# Autodesk Inventor assembly: final-print-(with_numbar)
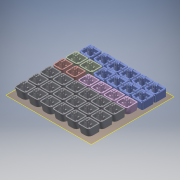
[picture p0: Inventor's stored thumbnail of the model, 180x180]
Saved by Autodesk Inventor 2018 (Build 220112000, 112)
## iProperties
Created: 2017-07-27
Part Number: final-print-(with_numbar)
Document SubType Name: Assembly
Designer: Jason Cemra
Author: Jason Cemra
## Documents named in this file (4)
- C:\Users\Jason Cemra\Documents\Logical Store\StenoToppers\stenotoppers\cherrymx\print-assemblies\final-print-(with_numbar).iam
- C:\Users\Jason Cemra\Documents\Logical Store\StenoToppers\stenotoppers\cherrymx\print-assemblies\final-print.iam
- C:\Users\Jason Cemra\Documents\Logical Store\StenoToppers\stenotoppers\cherrymx\stenotoppers\numbar_cmx.ipt
- C:\Users\Jason Cemra\Documents\Logical Store\StenoToppers\stenotoppers\cherrymx\stenotoppers.ipt
## Components (11 placed, 2 different names)
1. final-print:1 [sub-assembly] — Mate:1
2. numbar_cmx:9
3. numbar_cmx:1 — Mate:2
4. numbar_cmx:2
5. numbar_cmx:3
6. numbar_cmx:4
7. numbar_cmx:5
8. numbar_cmx:6
9. numbar_cmx:7
10. numbar_cmx:8
11. numbar_cmx:10
## Component patterns: (10 elements, first: numbar_cmx:1)
## Relationships (2: Mate 2)
- Mate:1: final-print:1
- Mate:2: numbar_cmx:1
